# Autodesk Inventor assembly: one side of tower
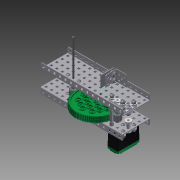
[picture p0: Inventor's stored thumbnail of the model, 180x180]
Saved by Autodesk Inventor 2014 SP1 (Build 180222100, 222)
## iProperties
Created: 2014-02-23
Part Number: one side of tower
Document SubType Name: Assembly
Designer: Ryan
Author: Ryan
## Documents named in this file (21)
- C:\Users\Ryan\Desktop\sw\toss up 4th robot\tower\one side of tower.iam
- C:\Users\Ryan\Desktop\sw\lib\Aperture VEX CAD Library\Metal\C Channel\5 x 15.ipt
- C:\Users\Ryan\Desktop\sw\lib\Aperture VEX CAD Library\Bearing Blocks\Bearing Block.ipt
- C:\Users\Ryan\Desktop\sw\lib\Aperture VEX CAD Library\Hardware\8-32\8-32 nylock.ipt
- C:\Users\Ryan\Desktop\sw\lib\Aperture VEX CAD Library\Hardware\8-32\8-32_.500.ipt
- C:\Users\Ryan\Desktop\sw\lib\Aperture VEX CAD Library\Spacers\thin\SPACER-0320-0125.ipt
- C:\Users\Ryan\Desktop\sw\lib\Aperture VEX CAD Library\Gears\High Strength Gears\HS-GEAR-12TOOTH.ipt
- C:\Users\Ryan\Desktop\sw\lib\Aperture VEX CAD Library\Spacers\thin\SPACER-0320-0500.ipt
- C:\Users\Ryan\Desktop\sw\lib\Aperture VEX CAD Library\Gears\High Strength Gears\Green HS 84.iam
- C:\Users\Ryan\Desktop\sw\lib\Aperture VEX CAD Library\Spacers\thin\SPACER-0320-0250.ipt
- C:\Users\Ryan\Desktop\sw\lib\Aperture VEX CAD Library\Hardware\Shaft Collar.ipt
- C:\Users\Ryan\Desktop\sw\lib\Aperture VEX CAD Library\Spacers\thin\SPACER-0320-0375.ipt
- C:\Users\Ryan\Desktop\sw\lib\Aperture VEX CAD Library\Standoffs\BEAM-1000.ipt
- C:\Users\Ryan\Desktop\sw\lib\Aperture VEX CAD Library\Hardware\8-32\8-32_.375.ipt
- C:\Users\Ryan\Desktop\sw\lib\Aperture VEX CAD Library\Standoffs\BEAM-0500.ipt
- C:\Users\Ryan\Desktop\sw\lib\Super Sonic Sparks VEX CAD Library\Motors & Sensors\2-Wire Motor 393-Without Wire.iam
- C:\Users\Ryan\Desktop\sw\lib\Aperture VEX CAD Library\Spacers\SPACER-0500-0250.ipt
- C:\Users\Ryan\Desktop\sw\lib\Aperture VEX CAD Library\Spacers\SPACER-0500-0625.ipt
- C:\Users\Ryan\Desktop\sw\lib\Aperture VEX CAD Library\Spacers\SPACER-0500-0125.ipt
- C:\Users\Ryan\Desktop\sw\lib\Aperture VEX CAD Library\Shaft\5.5 inch shaft.ipt
- C:\Users\Ryan\Desktop\sw\toss up 4th robot\tower\gyro asmb.iam
## Components (66 placed, 20 different names)
1. 5 x 15:1 — Flush:1, Flush:2, Mate:2, Mate:3, Mate:4, Mate:5, Mate:11, Mate:13, Flush:4, Mate:30, Mate:31, Mate:43, Mate:44, Mate:47, Mate:55, Mate:56, Mate:57, Mate:62, Mate:73, Mate:77, Mate:80, Mate:81, Mate:82, Mate:104, Mate:105, Mate:106, Mate:121, Mate:122, Mate:126, Mate:127
2. 5 x 15:2 — Flush:1, Flush:2, Flush:4, Mate:23, Mate:26, Mate:35, Mate:36, Mate:66, Mate:69, Mate:70, Mate:79, Mate:93, Mate:96, Mate:117, Mate:120, Mate:123, Mate:124, Mate:132, Mate:140, Mate:147, Flush:12, Flush:13
3. 8-32 nylock:1 — Mate:8, Mate:9, Mate:12
4. 8-32_.500:2 — Flush:3, Mate:12, Mate:95
5. 8-32_.500:1 — Mate:10, Mate:11, Flush:3
6. 8-32 nylock:2 — Mate:6, Mate:7, Mate:10
7. Bearing Block:1 — Mate:2, Mate:3, Mate:4, Mate:5, Mate:6, Mate:7, Mate:8, Mate:9, Mate:61, Mate:125
8. SPACER-0320-0125:1 — Mate:13, Mate:15, Mate:16, Mate:33
9. HS-GEAR-12TOOTH:1 — Mate:15, Mate:16, Mate:144, Mate:145
10. Bearing Block:4 — Mate:23, Mate:27, Mate:28, Mate:35, Mate:123
11. 8-32 nylock:7
12. 8-32 nylock:8
13. 8-32_.500:7 — Mate:26
14. 8-32_.500:8 — Mate:36
15. SPACER-0320-0500:1 — Mate:27, Mate:28, Mate:33, Mate:54
16. Green HS 84:1 [sub-assembly] — Mate:30, Mate:32, Mate:129
17. SPACER-0320-0125:2 — Mate:31, Mate:32, Mate:58
18. Bearing Block:5 — Mate:43, Mate:44, Mate:58
19. 8-32 nylock:9
20. 8-32 nylock:10
21. 8-32_.500:9 — Mate:122
22. 8-32_.500:10 — Mate:47, Mate:121
23. Bearing Block:6 — Mate:54, Mate:55, Flush:11
24. 8-32 nylock:11
25. 8-32 nylock:12 — Mate:56
26. 8-32_.500:11 — Mate:57
27. 8-32_.500:12
28. SPACER-0320-0125:3 — Mate:61, Mate:62, Mate:64
29. HS-GEAR-12TOOTH:2
30. SPACER-0320-0375:1 — Mate:64, Mate:65, Mate:146
31. SPACER-0320-0125:4 — Mate:65, Mate:66, Mate:67, Mate:68
32. Shaft Collar:1 — Mate:67, Mate:68, Mate:94, Mate:146
33. SPACER-0320-0125:5 — Mate:69, Mate:70, Mate:72, Mate:78, Mate:124
34. SPACER-0320-0250:1 — Mate:72, Mate:73, Mate:74, Mate:75, Mate:76
35. BEAM-1000:1 — Mate:74, Mate:75
36. 8-32_.500:13 — Mate:76, Mate:77
37. 8-32_.375:1 — Mate:78, Mate:79
38. BEAM-0500:1 — Mate:80, Mate:81, Mate:82, Mate:103, Mate:136
39. Bearing Block:7 — Mate:93, Mate:94, Mate:95
40. 8-32 nylock:13
41. 8-32 nylock:14
42. 8-32_.500:15
43. 8-32_.500:16 — Mate:96
44. Bearing Block:8 — Mate:103, Mate:104, Mate:107, Mate:108
45. 8-32 nylock:15
46. 8-32 nylock:16 — Mate:105
47. 8-32_.500:17 — Mate:106
48. 8-32_.500:18 — Mate:119
49. 8-32_.500:19 — Mate:107, Mate:108
50. Bearing Block:9 — Mate:117
51. 8-32 nylock:17
52. 8-32 nylock:18 — Mate:119
53. 8-32_.500:20
54. 8-32_.500:21 — Mate:120
55. 8-32_.500:22 — Mate:141
56. 2-Wire Motor 393-Without Wire:1 [sub-assembly] — Mate:125, Mate:126, Mate:127
57. Shaft Collar:2 — Mate:129, Mate:130, Mate:131, Mate:133, Mate:134
58. SPACER-0500-0250:1 — Mate:130, Mate:131
59. SPACER-0500-0625:1 — Mate:132, Mate:133, Mate:134
60. SPACER-0500-0125:1 — Mate:135, Mate:136, Mate:137
61. SPACER-0500-0625:2 — Mate:135, Mate:137
62. SPACER-0500-0125:2 — Mate:141, Mate:142, Mate:143
63. SPACER-0500-0625:3 — Mate:140
64. 8-32 nylock:19 — Mate:142, Mate:143
65. 5.5 inch shaft:1 — Mate:144, Flush:11, Mate:145
66. gyro asmb:1 [sub-assembly] — Mate:147, Flush:12, Flush:13
## Relationships (144: Mate 131, Flush 13)
- Flush:1: 5 x 15:1 ↔ 5 x 15:2
- Flush:2: 5 x 15:1 ↔ 5 x 15:2
- Mate:2: 5 x 15:1 ↔ Bearing Block:1
- Mate:3 (2.3114 mm): 5 x 15:1 ↔ Bearing Block:1
- Mate:4 (-48.4886 mm): 5 x 15:1 ↔ Bearing Block:1
- Mate:5 (53.1114 mm): 5 x 15:1 ↔ Bearing Block:1
- Mate:6: 8-32 nylock:2 ↔ Bearing Block:1
- Mate:7: 8-32 nylock:2 ↔ Bearing Block:1
- Mate:8: 8-32 nylock:1 ↔ Bearing Block:1
- Mate:9: 8-32 nylock:1 ↔ Bearing Block:1
- Mate:10: 8-32_.500:1 ↔ 8-32 nylock:2
- Mate:11: 5 x 15:1 ↔ 8-32_.500:1
- Flush:3: 8-32_.500:2 ↔ 8-32_.500:1
- Mate:12: 8-32 nylock:1 ↔ 8-32_.500:2
- Mate:13: 5 x 15:1 ↔ SPACER-0320-0125:1
- Mate:15: SPACER-0320-0125:1 ↔ HS-GEAR-12TOOTH:1
- Mate:16: SPACER-0320-0125:1 ↔ HS-GEAR-12TOOTH:1
- Flush:4 (50.8 mm): 5 x 15:1 ↔ 5 x 15:2
- [Mate]: Bearing Block:4 ↔ 8-32 nylock:8
- [Mate]: Bearing Block:4 ↔ 8-32 nylock:8
- [Mate]: Bearing Block:4 ↔ 8-32 nylock:7
- [Mate]: Bearing Block:4 ↔ 8-32 nylock:7
- [Mate]: 8-32 nylock:8 ↔ 8-32_.500:7
- [Flush]: 8-32_.500:7 ↔ 8-32_.500:8
- [Mate]: 8-32 nylock:7 ↔ 8-32_.500:8
- Mate:23: 5 x 15:2 ↔ Bearing Block:4
- Mate:26: 5 x 15:2 ↔ 8-32_.500:7
- Mate:27: Bearing Block:4 ↔ SPACER-0320-0500:1
- Mate:28: Bearing Block:4 ↔ SPACER-0320-0500:1
- Mate:30 (3.175 mm): 5 x 15:1 ↔ Green HS 84:1
- Mate:31: 5 x 15:1 ↔ SPACER-0320-0125:2
- Mate:32: Green HS 84:1 ↔ SPACER-0320-0125:2
- Mate:33: SPACER-0320-0125:1 ↔ SPACER-0320-0500:1
- Mate:35 (2.3114 mm): 5 x 15:2 ↔ Bearing Block:4
- Mate:36 (2.3114 mm): 5 x 15:2 ↔ 8-32_.500:8
- [Mate]: Bearing Block:5 ↔ 8-32 nylock:10
- [Mate]: Bearing Block:5 ↔ 8-32 nylock:10
- [Mate]: Bearing Block:5 ↔ 8-32 nylock:9
- [Mate]: Bearing Block:5 ↔ 8-32 nylock:9
- [Mate]: 8-32 nylock:10 ↔ 8-32_.500:9
- [Flush]: 8-32_.500:9 ↔ 8-32_.500:10
- [Mate]: 8-32 nylock:9 ↔ 8-32_.500:10
- Mate:43: 5 x 15:1 ↔ Bearing Block:5
- Mate:44 (2.3114 mm): 5 x 15:1 ↔ Bearing Block:5
- Mate:47: 5 x 15:1 ↔ 8-32_.500:10
- [Mate]: Bearing Block:6 ↔ 8-32 nylock:12
- [Mate]: Bearing Block:6 ↔ 8-32 nylock:12
- [Mate]: Bearing Block:6 ↔ 8-32 nylock:11
- [Mate]: Bearing Block:6 ↔ 8-32 nylock:11
- [Mate]: 8-32 nylock:12 ↔ 8-32_.500:11
- [Flush]: 8-32_.500:11 ↔ 8-32_.500:12
- [Mate]: 8-32 nylock:11 ↔ 8-32_.500:12
- Mate:54: SPACER-0320-0500:1 ↔ Bearing Block:6
- Mate:55: 5 x 15:1 ↔ Bearing Block:6
- Mate:56 (2.3114 mm): 5 x 15:1 ↔ 8-32 nylock:12
- Mate:57: 5 x 15:1 ↔ 8-32_.500:11
- Mate:58: SPACER-0320-0125:2 ↔ Bearing Block:5
- [Mate]: SPACER-0320-0125:3 ↔ HS-GEAR-12TOOTH:2
- [Mate]: SPACER-0320-0125:3 ↔ HS-GEAR-12TOOTH:2
- Mate:61: Bearing Block:1 ↔ SPACER-0320-0125:3
- Mate:62: 5 x 15:1 ↔ SPACER-0320-0125:3
- Mate:64: SPACER-0320-0125:3 ↔ SPACER-0320-0375:1
- Mate:65: SPACER-0320-0375:1 ↔ SPACER-0320-0125:4
- Mate:66: 5 x 15:2 ↔ SPACER-0320-0125:4
- Mate:67: SPACER-0320-0125:4 ↔ Shaft Collar:1
- Mate:68: SPACER-0320-0125:4 ↔ Shaft Collar:1
- Mate:69: 5 x 15:2 ↔ SPACER-0320-0125:5
- Mate:70 (2.3114 mm): 5 x 15:2 ↔ SPACER-0320-0125:5
- Mate:72: SPACER-0320-0125:5 ↔ SPACER-0320-0250:1
- Mate:73: 5 x 15:1 ↔ SPACER-0320-0250:1
- Mate:74: SPACER-0320-0250:1 ↔ BEAM-1000:1
- Mate:75: SPACER-0320-0250:1 ↔ BEAM-1000:1
- Mate:76: SPACER-0320-0250:1 ↔ 8-32_.500:13
- Mate:77: 5 x 15:1 ↔ 8-32_.500:13
- Mate:78: SPACER-0320-0125:5 ↔ 8-32_.375:1
- Mate:79: 5 x 15:2 ↔ 8-32_.375:1
- Mate:80: 5 x 15:1 ↔ BEAM-0500:1
- Mate:81 (2.3114 mm): 5 x 15:1 ↔ BEAM-0500:1
- Mate:82 (2.3114 mm): 5 x 15:1 ↔ BEAM-0500:1
- [Mate]: Bearing Block:7 ↔ 8-32 nylock:14
- [Mate]: Bearing Block:7 ↔ 8-32 nylock:14
- [Mate]: Bearing Block:7 ↔ 8-32 nylock:13
- [Mate]: Bearing Block:7 ↔ 8-32 nylock:13
- [Mate]: 8-32 nylock:14 ↔ 8-32_.500:15
- [Flush]: 8-32_.500:15 ↔ 8-32_.500:16
- [Mate]: 8-32 nylock:13 ↔ 8-32_.500:16
- Mate:93: 5 x 15:2 ↔ Bearing Block:7
- Mate:94: Shaft Collar:1 ↔ Bearing Block:7
- Mate:95: 8-32_.500:2 ↔ Bearing Block:7
- Mate:96: 5 x 15:2 ↔ 8-32_.500:16
- [Mate]: Bearing Block:8 ↔ 8-32 nylock:16
- [Mate]: Bearing Block:8 ↔ 8-32 nylock:16
- [Mate]: Bearing Block:8 ↔ 8-32 nylock:15
- [Mate]: Bearing Block:8 ↔ 8-32 nylock:15
- [Mate]: 8-32 nylock:16 ↔ 8-32_.500:17
- [Flush]: 8-32_.500:17 ↔ 8-32_.500:18
- [Mate]: 8-32 nylock:15 ↔ 8-32_.500:18
- Mate:103: BEAM-0500:1 ↔ Bearing Block:8
- Mate:104: 5 x 15:1 ↔ Bearing Block:8
- Mate:105 (2.3114 mm): 5 x 15:1 ↔ 8-32 nylock:16
- Mate:106: 5 x 15:1 ↔ 8-32_.500:17
- Mate:107: Bearing Block:8 ↔ 8-32_.500:19
- Mate:108: Bearing Block:8 ↔ 8-32_.500:19
- [Mate]: Bearing Block:9 ↔ 8-32 nylock:18
- [Mate]: Bearing Block:9 ↔ 8-32 nylock:18
- [Mate]: Bearing Block:9 ↔ 8-32 nylock:17
- [Mate]: Bearing Block:9 ↔ 8-32 nylock:17
- [Mate]: 8-32 nylock:18 ↔ 8-32_.500:20
- [Flush]: 8-32_.500:20 ↔ 8-32_.500:21
- [Mate]: 8-32 nylock:17 ↔ 8-32_.500:21
- [Mate]: Bearing Block:9 ↔ 8-32_.500:22
- [Mate]: Bearing Block:9 ↔ 8-32_.500:22
- Mate:117: 5 x 15:2 ↔ Bearing Block:9
- Mate:119: 8-32_.500:18 ↔ 8-32 nylock:18
- Mate:120: 5 x 15:2 ↔ 8-32_.500:21
- Mate:121 (2.3114 mm): 5 x 15:1 ↔ 8-32_.500:10
- Mate:122 (2.3114 mm): 5 x 15:1 ↔ 8-32_.500:9
- Mate:123 (2.3114 mm): 5 x 15:2 ↔ Bearing Block:4
- Mate:124 (2.3114 mm): 5 x 15:2 ↔ SPACER-0320-0125:5
- Mate:125: Bearing Block:1 ↔ 2-Wire Motor 393-Without Wire:1
- Mate:126: 5 x 15:1 ↔ 2-Wire Motor 393-Without Wire:1
- Mate:127 (2.3114 mm): 5 x 15:1 ↔ 2-Wire Motor 393-Without Wire:1
- Mate:129: Green HS 84:1 ↔ Shaft Collar:2
- Mate:130: Shaft Collar:2 ↔ SPACER-0500-0250:1
- Mate:131: Shaft Collar:2 ↔ SPACER-0500-0250:1
- Mate:132: 5 x 15:2 ↔ SPACER-0500-0625:1
- Mate:133: Shaft Collar:2 ↔ SPACER-0500-0625:1
- Mate:134: Shaft Collar:2 ↔ SPACER-0500-0625:1
- Mate:135: SPACER-0500-0125:1 ↔ SPACER-0500-0625:2
- Mate:136: BEAM-0500:1 ↔ SPACER-0500-0125:1
- Mate:137: SPACER-0500-0125:1 ↔ SPACER-0500-0625:2
- [Mate]: SPACER-0500-0125:2 ↔ SPACER-0500-0625:3
- [Mate]: SPACER-0500-0125:2 ↔ SPACER-0500-0625:3
- Mate:140: 5 x 15:2 ↔ SPACER-0500-0625:3
- Mate:141: 8-32_.500:22 ↔ SPACER-0500-0125:2
- Mate:142: SPACER-0500-0125:2 ↔ 8-32 nylock:19
- Mate:143: SPACER-0500-0125:2 ↔ 8-32 nylock:19
- Mate:144: HS-GEAR-12TOOTH:1 ↔ 5.5 inch shaft:1
- Flush:11: Bearing Block:6 ↔ 5.5 inch shaft:1
- Mate:145: HS-GEAR-12TOOTH:1 ↔ 5.5 inch shaft:1
- Mate:146: SPACER-0320-0375:1 ↔ Shaft Collar:1
- Mate:147: 5 x 15:2 ↔ gyro asmb:1
- Flush:12: 5 x 15:2 ↔ gyro asmb:1
- Flush:13: 5 x 15:2 ↔ gyro asmb:1
## Named parameters: q = 2.3114 mm, d25_d7 = 0 mm, d26_d8 = 0 mm, d27_d9 = 0 mm, d28_d10 = 0 mm, d29_d11 = 0 mm, d30_d13 = 0 mm, d31_d14 = 0 mm, d47_d7 = 0 mm, d48_d8 = 0 mm, d49_d9 = 0 mm, d50_d10 = 0 mm, d51_d11 = 0 mm, d52_d13 = 0 mm, d53_d14 = 0 mm, d59_d7 = 0 mm, d60_d8 = 0 mm, d61_d9 = 0 mm, d62_d10 = 0 mm, d63_d11 = 0 mm, d64_d13 = 0 mm, d65_d14 = 0 mm, d71_d21 = 0 mm, d72_d22 = 0 mm, d99_d7 = 0 mm, d100_d8 = 0 mm, d101_d9 = 0 mm, d102_d10 = 0 mm, d103_d11 = 0 mm, d104_d13 = 0 mm, d105_d14 = 0 mm, d110_d7 = 0 mm, d111_d8 = 0 mm, d112_d9 = 0 mm, d113_d10 = 0 mm, d114_d11 = 0 mm, d115_d13 = 0 mm, d116_d14 = 0 mm, d123_d110_d7 = 0 mm, d124_d111_d8 = 0 mm, d125_d112_d9 = 0 mm, d126_d113_d10 = 0 mm, d127_d114_d11 = 0 mm, d128_d115_d13 = 0 mm, d129_d116_d14 = 0 mm, d130_d121 = 0 mm, d131_d122 = 0 mm, d153_d150 = 0 mm, d154_d152 = 0 mm
